# Autodesk Inventor assembly: IFI-WHEEL-ASSY-815-50
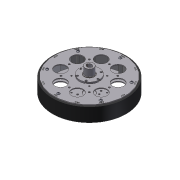
[picture p0: Inventor's stored thumbnail of the model, 180x180]
Saved by Autodesk Inventor 2012 (Build 160160000, 160)
## iProperties
Created: 2012-01-24
Part Number: IFI-WHEEL-ASSY-815-50
Document SubType Name: Assembly
Designer: JesseK
Mass: 2197.4 g
Surface Area: 3409.94 cm^2
Volume: 958.094 cm^3
Density: 2.29351 g/cm^3
Translation Standard: STEP AP203
FileName: IFI-WHEEL-ASSY-815-50.STEP
PreProcessor: SolidWorks 2006052
PostProcessor: Build: 160, Release: 2012 RTM - Date: Tue 03/01/2011
Sent Units: inch
Uncertainty: 1e-05
Author: JesseK
## Documents named in this file (7)
- Z:\UserData\Documents\Inventor\team1885frc\IFI\Imported Components\IFI-WHEEL-ASSY-815-50\IFI-WHEEL-ASSY-815-50.iam
- Z:\UserData\Documents\Inventor\team1885frc\IFI\Imported Components\IFI-WHEEL-ASSY-815-50\TB-WHEEL-RIM-815 RevG.ipt
- Z:\UserData\Documents\Inventor\team1885frc\IFI\Imported Components\IFI-WHEEL-ASSY-815-50\SBS_SBS0832-0500SS.ipt
- Z:\UserData\Documents\Inventor\team1885frc\IFI\Imported Components\IFI-WHEEL-ASSY-815-50\THF0832-0250-1500.ipt
- Z:\UserData\Documents\Inventor\team1885frc\IFI\Imported Components\IFI-WHEEL-ASSY-815-50\TB-WHEEL-HUB-850 RevG.ipt
- Z:\UserData\Documents\Inventor\team1885frc\IFI\Imported Components\IFI-WHEEL-ASSY-815-50\8x15.ipt
- Z:\UserData\Documents\Inventor\team1885frc\AndyMark\500EX-Key-Hub.ipt
## Components (26 placed, 6 different names)
1. TB-WHEEL-RIM-815 RevG:1
2. SBS_SBS0832-0500SS:1
3. SBS_SBS0832-0500SS:3
4. THF0832-0250-1500:1
5. SBS_SBS0832-0500SS:4
6. SBS_SBS0832-0500SS:5
7. THF0832-0250-1500:2
8. THF0832-0250-1500:3
9. TB-WHEEL-HUB-850 RevG:1 — Mate:14, Mate:15
10. SBS_SBS0832-0500SS:7
11. SBS_SBS0832-0500SS:8
12. THF0832-0250-1500:4
13. SBS_SBS0832-0500SS:9
14. SBS_SBS0832-0500SS:10
15. SBS_SBS0832-0500SS:11
16. TB-WHEEL-RIM-815 RevG:2
17. SBS_SBS0832-0500SS:12
18. THF0832-0250-1500:5
19. TB-WHEEL-HUB-850 RevG:2 — Mate:13, Mate:16
20. TB-WHEEL-RIM-815 RevG:3
21. SBS_SBS0832-0500SS:13
22. THF0832-0250-1500:6
23. 8x15:1
24. SBS_SBS0832-0500SS:16
25. 500EX-Key-Hub:1 — Mate:13, Mate:16
26. 500EX-Key-Hub:2 — Mate:14, Mate:15
## Relationships (4: Mate 4)
- Mate:13: TB-WHEEL-HUB-850 RevG:2 ↔ 500EX-Key-Hub:1
- Mate:14: TB-WHEEL-HUB-850 RevG:1 ↔ 500EX-Key-Hub:2
- Mate:15: TB-WHEEL-HUB-850 RevG:1 ↔ 500EX-Key-Hub:2
- Mate:16: TB-WHEEL-HUB-850 RevG:2 ↔ 500EX-Key-Hub:1
